# Autodesk Inventor assembly: glue
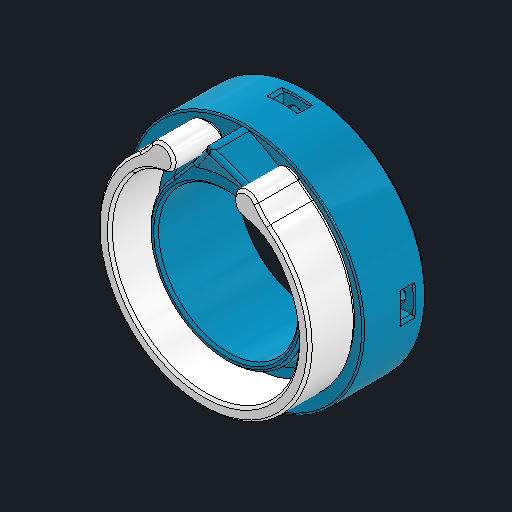
[picture p0: Inventor's stored thumbnail of the model, 512x512]
Saved by Autodesk Inventor 2026 (Build 300175050, 175E)
## iProperties
Created: 2026-01-07
Part Number: glue
Document SubType Name: Assembly
Designer: queezz
Author: queezz
## Documents named in this file (3)
- C:\Users\queezz\Dropbox\Drawings\PIHTI\3D-printing\glue.iam
- C:\Users\queezz\Dropbox\Drawings\PIHTI\PLD\pld-octogon-nipple.ipt
- C:\Users\queezz\Dropbox\Drawings\PIHTI\PLD\glue-support-port.ipt
## Components (2 placed, 2 different names)
1. pld-octogon-nipple:1 — Mate:1, Tangent:1
2. glue-support-port:1 — Mate:1, Tangent:1
## Relationships (2: Mate 1, Tangent 1)
- Mate:1: pld-octogon-nipple:1 ↔ glue-support-port:1
- Tangent:1: pld-octogon-nipple:1 ↔ glue-support-port:1
